# Autodesk Inventor assembly: LEG2
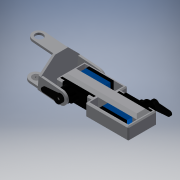
[picture p0: Inventor's stored thumbnail of the model, 180x180]
Saved by Autodesk Inventor 2017 (Build 210142000, 142)
## iProperties
Created: 2017-09-24
Part Number: LEG2
Document SubType Name: Assembly
Designer: Alexander Miller
Author: Alexander Miller
## Documents named in this file (6)
- D:\Daten\Documents\Git\HeRo-Mini\Hardware\LEG.iam
- D:\Daten\Documents\Git\HeRo-Mini\Hardware\SERVO.iam
- D:\Daten\Documents\Git\HeRo-Mini\Hardware\COXA.ipt
- D:\Daten\Documents\Git\HeRo-Mini\Hardware\FEMUR_A.ipt
- D:\Daten\Documents\Git\HeRo-Mini\Hardware\FEMUR_B.ipt
- D:\Daten\Documents\Git\HeRo-Mini\Hardware\BEARING.ipt
## Components (8 placed, 5 different names)
1. SERVO:1 [sub-assembly] — Rigid:1, Rigid:3, Rigid:5
2. SERVO:2 [sub-assembly] — Rigid:2, Rigid:4
3. COXA:1 — Rigid:5, Rotational:1, Rotational:2
4. FEMUR_A:1 — Rigid:1, Rigid:2
5. FEMUR_B:1 — Rigid:4
6. FEMUR_B:2 — Rigid:3
7. BEARING:1 — Rotational:1
8. BEARING:2 — Rotational:2
## Relationships (7: WeldJoint 5, RevoluteJoint 2)
- Rigid:1 [WeldJoint]: SERVO:1 ↔ FEMUR_A:1
- Rigid:2 [WeldJoint]: SERVO:2 ↔ FEMUR_A:1
- Rigid:3 [WeldJoint]: SERVO:1 ↔ FEMUR_B:2
- Rigid:4 [WeldJoint]: SERVO:2 ↔ FEMUR_B:1
- Rigid:5 [WeldJoint]: SERVO:1 ↔ COXA:1
- Rotational:1 [RevoluteJoint]: COXA:1 ↔ BEARING:1
- Rotational:2 [RevoluteJoint]: COXA:1 ↔ BEARING:2
